# Autodesk Inventor assembly: Turdbot Drivetrain
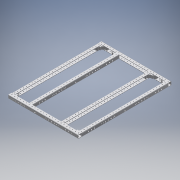
[picture p0: Inventor's stored thumbnail of the model, 180x180]
Saved by Autodesk Inventor 2016 (Build 200138000, 138)
## iProperties
Created: 2016-01-13
Part Number: Turdbot Drivetrain
Document SubType Name: Assembly
Designer: Administrator
Author: Administrator
## Documents named in this file (3)
- C:\Users\Administrator\Desktop\3192CAD\InitialRobotProto\Turdbot Drivetrain.iam
- C:\Users\Administrator\Desktop\3192CAD\InitialRobotProto\DBK_C-Channel_am-2222.ipt
- C:\Users\Administrator\Desktop\3192CAD\InitialRobotProto\DBK_CornerConnect_am-0212.ipt
## Components (12 placed, 2 different names)
1. DBK_C-Channel_am-2222:1 — Mate:1, Mate:2, Mate:3, Mate:16, Mate:17, Mate:18
2. DBK_C-Channel_am-2222:2 — Mate:4, Mate:5, Mate:6, Mate:7, Mate:8, Mate:9, Mate:22, Mate:23, Mate:24, Mate:25, Mate:26, Mate:27
3. DBK_C-Channel_am-2222:3 — Mate:19, Mate:20, Mate:21
4. DBK_C-Channel_am-2222:4 — Mate:10, Mate:11, Mate:12, Mate:13, Mate:14, Mate:15
5. DBK_CornerConnect_am-0212:1 — Mate:7, Mate:8, Mate:9, Mate:10, Mate:11, Mate:12
6. DBK_CornerConnect_am-0212:2 — Mate:16, Mate:17, Mate:18
7. DBK_CornerConnect_am-0212:3 — Mate:1, Mate:2, Mate:3, Mate:4, Mate:5, Mate:6
8. DBK_CornerConnect_am-0212:4 — Mate:13, Mate:14, Mate:15, Mate:19, Mate:20, Mate:21
9. DBK_C-Channel_am-2222:5 — Mate:31, Mate:32, Mate:33
10. DBK_C-Channel_am-2222:6 — Mate:28, Mate:29, Mate:30
11. DBK_CornerConnect_am-0212:5 — Mate:22, Mate:23, Mate:24, Mate:31, Mate:32, Mate:33
12. DBK_CornerConnect_am-0212:6 — Mate:25, Mate:26, Mate:27, Mate:28, Mate:29, Mate:30
## Relationships (33: Mate 33)
- Mate:1: DBK_C-Channel_am-2222:1 ↔ DBK_CornerConnect_am-0212:3
- Mate:2: DBK_C-Channel_am-2222:1 ↔ DBK_CornerConnect_am-0212:3
- Mate:3: DBK_C-Channel_am-2222:1 ↔ DBK_CornerConnect_am-0212:3
- Mate:4: DBK_C-Channel_am-2222:2 ↔ DBK_CornerConnect_am-0212:3
- Mate:5: DBK_C-Channel_am-2222:2 ↔ DBK_CornerConnect_am-0212:3
- Mate:6: DBK_C-Channel_am-2222:2 ↔ DBK_CornerConnect_am-0212:3
- Mate:7: DBK_C-Channel_am-2222:2 ↔ DBK_CornerConnect_am-0212:1
- Mate:8: DBK_C-Channel_am-2222:2 ↔ DBK_CornerConnect_am-0212:1
- Mate:9: DBK_C-Channel_am-2222:2 ↔ DBK_CornerConnect_am-0212:1
- Mate:10: DBK_C-Channel_am-2222:4 ↔ DBK_CornerConnect_am-0212:1
- Mate:11: DBK_C-Channel_am-2222:4 ↔ DBK_CornerConnect_am-0212:1
- Mate:12: DBK_C-Channel_am-2222:4 ↔ DBK_CornerConnect_am-0212:1
- Mate:13: DBK_C-Channel_am-2222:4 ↔ DBK_CornerConnect_am-0212:4
- Mate:14: DBK_C-Channel_am-2222:4 ↔ DBK_CornerConnect_am-0212:4
- Mate:15: DBK_C-Channel_am-2222:4 ↔ DBK_CornerConnect_am-0212:4
- Mate:16: DBK_C-Channel_am-2222:1 ↔ DBK_CornerConnect_am-0212:2
- Mate:17: DBK_C-Channel_am-2222:1 ↔ DBK_CornerConnect_am-0212:2
- Mate:18: DBK_C-Channel_am-2222:1 ↔ DBK_CornerConnect_am-0212:2
- Mate:19: DBK_C-Channel_am-2222:3 ↔ DBK_CornerConnect_am-0212:4
- Mate:20: DBK_C-Channel_am-2222:3 ↔ DBK_CornerConnect_am-0212:4
- Mate:21: DBK_C-Channel_am-2222:3 ↔ DBK_CornerConnect_am-0212:4
- Mate:22: DBK_C-Channel_am-2222:2 ↔ DBK_CornerConnect_am-0212:5
- Mate:23: DBK_C-Channel_am-2222:2 ↔ DBK_CornerConnect_am-0212:5
- Mate:24: DBK_C-Channel_am-2222:2 ↔ DBK_CornerConnect_am-0212:5
- Mate:25: DBK_C-Channel_am-2222:2 ↔ DBK_CornerConnect_am-0212:6
- Mate:26: DBK_C-Channel_am-2222:2 ↔ DBK_CornerConnect_am-0212:6
- Mate:27: DBK_C-Channel_am-2222:2 ↔ DBK_CornerConnect_am-0212:6
- Mate:28: DBK_C-Channel_am-2222:6 ↔ DBK_CornerConnect_am-0212:6
- Mate:29: DBK_C-Channel_am-2222:6 ↔ DBK_CornerConnect_am-0212:6
- Mate:30: DBK_C-Channel_am-2222:6 ↔ DBK_CornerConnect_am-0212:6
- Mate:31: DBK_C-Channel_am-2222:5 ↔ DBK_CornerConnect_am-0212:5
- Mate:32: DBK_C-Channel_am-2222:5 ↔ DBK_CornerConnect_am-0212:5
- Mate:33: DBK_C-Channel_am-2222:5 ↔ DBK_CornerConnect_am-0212:5
